# Autodesk Inventor assembly: 551373 SMT-10M-PS-24V-E-2,5-L-OE
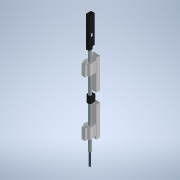
[picture p0: Inventor's stored thumbnail of the model, 180x180]
Saved by Autodesk Inventor 2021 (Build 250183000, 183)
## iProperties
Category: PARTsolutions
Company: FESTO
Created: 2025-06-05
Part Number: 551373 SMT-10M-PS-24V-E-2,5-L-OE
Catalog Web Link: www.cadenas.de
Description: SMT-10M-proximity sensor
Vendor: FESTO
Document SubType Name: Assembly
Designer: psAdmin
Manufacturer: FESTO
Mass: 16.8 g
Surface Area: 32.7923 cm^2
Volume: 1.15115 cm^3
Density: 14.5941 g/cm^3
Title: 551373 SMT-10M-PS-24V-E-2,5-L-OE
Author: Cadenas PARTsolutions
Comments: proximity sensor
PSOL_IDENT_0: {ATYP=ASSISTANT},{DATA=script=$CADENAS_DATA/23d-libs/festo/webfesto.vbb&M_FAMILY=SMT&M_GROUP=01&M_PA
PSOL_IDENT_1: RTNO=551373&IDCODE1=SMT-10M-PS-24V-E-25-L-OE&IDCODE2=&customer_number_cns=&MATES=1&LOD=HI&LOCKERP=0&
PSOL_IDENT_2: SINGLEPART=1}
NB: 551373 SMT-10M-PS-24V-E-2,5-L-OE
NN: SMT-10M
NT: proximity sensor
NBSYN: $TNR. $TYP.
LINA: 551373 SMT-10M-PS-24V-E-2,5-L-OE
CATALOG: Festo
TNR: 551373
TYP: SMT-10M-PS-24V-E-2,5-L-OE
B1: 2.95
D1: 2.15
D2: -
D3: 0
H1: 4.6
L1: 2.5
L2: 50
L3: 22.95
L4: 20.95
L5: 23
L6: 7
SW: 1.5
CNSMASSEXACT: 0.0168
GTIN: 4052568094737
SUPPLIER: FESTO
ARTICLENO: 551373 SMT-10M-PS-24V-E-2,5-L-OE
BOMINFO: 551373 SMT-10M-PS-24V-E-2,5-L-OE
CREATOR: CADENAS GmbH
## Documents named in this file (4)
- e:\temp\worker_COMMON_227\temp\tmp_3020_14_1dd7H\format_0\551373 SMT-10M-PS-24V-E-2,5-L-OE.iam
- e:\temp\worker_COMMON_227\temp\tmp_3020_14_1dd7H\format_0\551373 SMT-10M-PS-24V-E-2_5-L-OE.ipt
- e:\temp\worker_COMMON_227\temp\tmp_3020_14_1dd7H\format_0\1247168 ASCF-M-23-S DM 2_1-3_4.ipt
- e:\temp\worker_COMMON_227\temp\tmp_3020_14_1dd7H\format_0\534255 SMBK-10.ipt
## Components (4 placed, 3 different names)
1. 551373 SMT-10M-PS-24V-E-2_5-L-OE:1 — ASCF1_XY@1 <-> KTN_XY@2, ASCF1_Z@1 <-> KTN_Z@2, ASCF1_YZ@1 <-> KTN_YZ@2, ASCF2_XY@1 <-> KTN_XY@3, ASCF2_Z@1 <-> KTN_Z@3, ASCF2_YZ@1 <-> KTN_YZ@3, CLIP_XY@1 <-> ANBAU_XY@4, CLIP_Z@1 <-> ANBAU_Z@4, CLIP_YZ@1 <-> ANBAU_YZ@4
2. 1247168 ASCF-M-23-S DM 2_1-3_4:1 — ASCF1_XY@1 <-> KTN_XY@2, ASCF1_Z@1 <-> KTN_Z@2, ASCF1_YZ@1 <-> KTN_YZ@2
3. 1247168 ASCF-M-23-S DM 2_1-3_4:2 — ASCF2_XY@1 <-> KTN_XY@3, ASCF2_Z@1 <-> KTN_Z@3, ASCF2_YZ@1 <-> KTN_YZ@3
4. 534255 SMBK-10:1 — CLIP_XY@1 <-> ANBAU_XY@4, CLIP_Z@1 <-> ANBAU_Z@4, CLIP_YZ@1 <-> ANBAU_YZ@4
## Relationships (9: Mate 6, Angle 3)
- ASCF1_XY@1 <-> KTN_XY@2 [Mate]: 551373 SMT-10M-PS-24V-E-2_5-L-OE:1 ↔ 1247168 ASCF-M-23-S DM 2_1-3_4:1
- ASCF1_Z@1 <-> KTN_Z@2 [Mate]: 551373 SMT-10M-PS-24V-E-2_5-L-OE:1 ↔ 1247168 ASCF-M-23-S DM 2_1-3_4:1
- ASCF1_YZ@1 <-> KTN_YZ@2 [Angle] (0 deg): 551373 SMT-10M-PS-24V-E-2_5-L-OE:1 ↔ 1247168 ASCF-M-23-S DM 2_1-3_4:1
- ASCF2_XY@1 <-> KTN_XY@3 [Mate]: 551373 SMT-10M-PS-24V-E-2_5-L-OE:1 ↔ 1247168 ASCF-M-23-S DM 2_1-3_4:2
- ASCF2_Z@1 <-> KTN_Z@3 [Mate]: 551373 SMT-10M-PS-24V-E-2_5-L-OE:1 ↔ 1247168 ASCF-M-23-S DM 2_1-3_4:2
- ASCF2_YZ@1 <-> KTN_YZ@3 [Angle] (180 deg): 551373 SMT-10M-PS-24V-E-2_5-L-OE:1 ↔ 1247168 ASCF-M-23-S DM 2_1-3_4:2
- CLIP_XY@1 <-> ANBAU_XY@4 [Mate]: 551373 SMT-10M-PS-24V-E-2_5-L-OE:1 ↔ 534255 SMBK-10:1
- CLIP_Z@1 <-> ANBAU_Z@4 [Mate]: 551373 SMT-10M-PS-24V-E-2_5-L-OE:1 ↔ 534255 SMBK-10:1
- CLIP_YZ@1 <-> ANBAU_YZ@4 [Angle] (0 deg): 551373 SMT-10M-PS-24V-E-2_5-L-OE:1 ↔ 534255 SMBK-10:1
